# Autodesk Inventor assembly: vacuum-nozzle-assembly
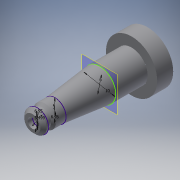
[picture p0: Inventor's stored thumbnail of the model, 180x180]
Saved by Autodesk Inventor 2017 (Build 210142000, 142)
## iProperties
Created: 2026-03-25
Part Number: vacuum-nozzle-assembly
Document SubType Name: Assembly
Designer: a
Author: a
## Documents named in this file (3)
- C:\Users\a\Documents\the-claw-pnp\vacuum-nozzle-assembly.iam
- C:\Users\a\Documents\the-claw-pnp\vacuum-nozzle-shaft.ipt
- C:\Users\a\Documents\the-claw-pnp\juki-mount.ipt
## Components (2 placed, 2 different names)
1. vacuum-nozzle-shaft:1 — Mate:1, Mate:2
2. juki-mount:1 — Mate:1, Mate:2
## Relationships (2: Mate 2)
- Mate:1: vacuum-nozzle-shaft:1 ↔ juki-mount:1
- Mate:2: vacuum-nozzle-shaft:1 ↔ juki-mount:1
